# Autodesk Inventor assembly: YaxisAss
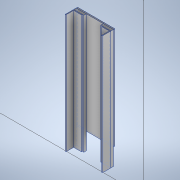
[picture p0: Inventor's stored thumbnail of the model, 180x180]
Saved by Autodesk Inventor 2022 (Build 260153000, 153)
## iProperties
Created: 2023-08-15
Part Number: YaxisAss
Document SubType Name: Assembly
Designer: Kippi
Author: Kippi
## Documents named in this file (4)
- C:\Users\Kippi\Documents\CNC_Lathe\YaxisAss.iam
- C:\Users\Kippi\Documents\CNC_Lathe\PodkladkaY.ipt
- C:\Users\Kippi\Documents\CNC_Lathe\Ugol700.ipt
- C:\Users\Kippi\Documents\CNC_Lathe\AxisY.ipt
## Components (5 placed, 3 different names)
1. PodkladkaY:1 — Mate:1, Flush:3, Flush:4, Mate:3, Flush:6
2. Ugol700:1 — Mate:3, Flush:5, Flush:6
3. PodkladkaY:2 — Mate:2, Flush:1, Flush:2, Mate:4, Flush:7, Flush:8
4. Ugol700:2 — Mate:4, Flush:7, Flush:8
5. AxisY:1 — Mate:1, Mate:2, Flush:1, Flush:2, Flush:3, Flush:4, Flush:5
## Relationships (12: Flush 8, Mate 4)
- Mate:1: PodkladkaY:1 ↔ AxisY:1
- Mate:2: PodkladkaY:2 ↔ AxisY:1
- Flush:1: PodkladkaY:2 ↔ AxisY:1
- Flush:2: PodkladkaY:2 ↔ AxisY:1
- Flush:3: PodkladkaY:1 ↔ AxisY:1
- Flush:4: PodkladkaY:1 ↔ AxisY:1
- Mate:3: PodkladkaY:1 ↔ Ugol700:1
- Flush:5: Ugol700:1 ↔ AxisY:1
- Flush:6: PodkladkaY:1 ↔ Ugol700:1
- Mate:4: PodkladkaY:2 ↔ Ugol700:2
- Flush:7: PodkladkaY:2 ↔ Ugol700:2
- Flush:8: PodkladkaY:2 ↔ Ugol700:2
